# Autodesk Inventor assembly: Assembly1
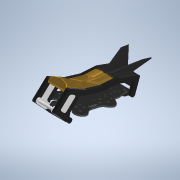
[picture p0: Inventor's stored thumbnail of the model, 180x180]
Saved by Autodesk Inventor 2020 (Build 240168000, 168)
## iProperties
Created: 2022-05-03
Part Number: Assembly1
Document SubType Name: Assembly
Designer: Steven
Author: Steven
## Documents named in this file (11)
- Y:\FPV drone stuff\0 Street League\Frames\PB-Kauri-X\3D prints\35 mm canopy\Assembly1.iam
- Y:\FPV drone stuff\0 Street League\Frames\PB-Kauri-X\Kauri side plate.ipt
- Y:\FPV drone stuff\0 Street League\Frames\PB-Kauri-X\3D prints\35 mm canopy\KauriCanopy Pb.ipt
- Y:\FPV drone stuff\0 Street League\Frames\PB-Kauri-X\3D prints\35 mm canopy\Spoiler v13 35mm.ipt
- Y:\FPV drone stuff\0 Street League\Frames\PB-Kauri-X\3D prints\KauriSpoilerFin.ipt
- Y:\FPV drone stuff\0 Street League\Frames\PB-Kauri-X\Kauri mid plate v2.ipt
- Y:\FPV drone stuff\0 Street League\Frames\PB-Kauri-X\3D prints\35 mm canopy\KauriFrontLink 35mm.ipt
- Y:\FPV drone stuff\0 Street League\Frames\PB-Kauri-X\3D prints\35 mm canopy\KauriRearLink 35mm no brass insert.ipt
- Y:\FPV drone stuff\0 Street League\Frames\PB-Kauri-X\3D prints\35 mm canopy\Kauri camera mount.ipt
- Y:\FPV drone stuff\0 Street League\Frames\PB-Kauri-X\3D prints\35 mm canopy\35mm standoff.ipt
- Y:\FPV drone stuff\0 Street League\Frames\PB-Kauri-X\3D prints\35 mm canopy\Kauri camera mount mirror.ipt
## Components (12 placed, 10 different names)
1. Kauri side plate:1 — Mate:1, Insert:3, Insert:4, Mate:4, Insert:12, Insert:15, Insert:16, Insert:20, Insert:21
2. KauriCanopy Pb:1 — Mate:1, Insert:3, Insert:4, Mate:9, Insert:13, Insert:14
3. Spoiler v13 35mm:1 — Mate:4, Insert:7, Mate:5, Insert:15, Insert:16
4. KauriSpoilerFin:1 — Insert:7, Mate:5
5. Kauri mid plate v2:1 — Mate:6, Insert:8, Mate:7, Mate:8, Insert:10, Insert:11
6. KauriFrontLink 35mm:1 — Mate:6, Insert:8, Mate:7, Insert:17
7. KauriRearLink 35mm no brass insert:1 — Mate:8, Insert:10, Insert:11, Insert:12
8. Kauri side plate:2 — Mate:9, Insert:13, Insert:14, Mate:10, Mate:11, Mate:12, Insert:17, Insert:18, Insert:19
9. Kauri camera mount:1 — Mate:10, Mate:11, Mate:12
10. 35mm standoff:1 — Insert:18
11. 35mm standoff:2 — Insert:19
12. Kauri camera mount mirror:1 — Insert:20, Insert:21
## Relationships (26: Insert 16, Mate 10)
- Mate:1: Kauri side plate:1 ↔ KauriCanopy Pb:1
- Insert:3: Kauri side plate:1 ↔ KauriCanopy Pb:1
- Insert:4: Kauri side plate:1 ↔ KauriCanopy Pb:1
- Mate:4: Kauri side plate:1 ↔ Spoiler v13 35mm:1
- Insert:7: Spoiler v13 35mm:1 ↔ KauriSpoilerFin:1
- Mate:5: Spoiler v13 35mm:1 ↔ KauriSpoilerFin:1
- Mate:6: Kauri mid plate v2:1 ↔ KauriFrontLink 35mm:1
- Insert:8: Kauri mid plate v2:1 ↔ KauriFrontLink 35mm:1
- Mate:7: Kauri mid plate v2:1 ↔ KauriFrontLink 35mm:1
- Mate:8: Kauri mid plate v2:1 ↔ KauriRearLink 35mm no brass insert:1
- Insert:10: Kauri mid plate v2:1 ↔ KauriRearLink 35mm no brass insert:1
- Insert:11: Kauri mid plate v2:1 ↔ KauriRearLink 35mm no brass insert:1
- Insert:12: Kauri side plate:1 ↔ KauriRearLink 35mm no brass insert:1
- Mate:9: KauriCanopy Pb:1 ↔ Kauri side plate:2
- Insert:13: KauriCanopy Pb:1 ↔ Kauri side plate:2
- Insert:14: KauriCanopy Pb:1 ↔ Kauri side plate:2
- Insert:15: Kauri side plate:1 ↔ Spoiler v13 35mm:1
- Mate:10: Kauri side plate:2 ↔ Kauri camera mount:1
- Mate:11: Kauri side plate:2 ↔ Kauri camera mount:1
- Mate:12: Kauri side plate:2 ↔ Kauri camera mount:1
- Insert:16: Kauri side plate:1 ↔ Spoiler v13 35mm:1
- Insert:17: KauriFrontLink 35mm:1 ↔ Kauri side plate:2
- Insert:18: Kauri side plate:2 ↔ 35mm standoff:1
- Insert:19: Kauri side plate:2 ↔ 35mm standoff:2
- Insert:20: Kauri side plate:1 ↔ Kauri camera mount mirror:1
- Insert:21: Kauri side plate:1 ↔ Kauri camera mount mirror:1
